# Autodesk Inventor assembly: 라즈베리파이 조립품
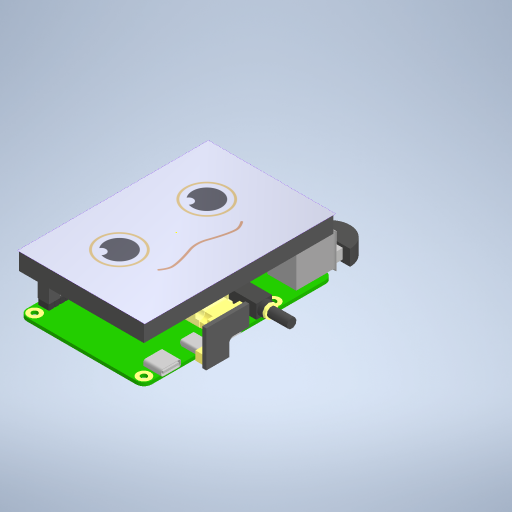
[picture p0: Inventor's stored thumbnail of the model, 512x512]
Saved by Autodesk Inventor 2023 (Build 270158000, 158)
## iProperties
Created: 2022-08-09
Part Number: 라즈베리파이 조립품
Document SubType Name: Assembly
Designer: fly01
Author: fly01
## Documents named in this file (6)
- C:\Users\user\Desktop\PAI\PAI설계\조림품\라즈베리파이 조립품.iam
- C:\Users\user\Desktop\PAI\PAI설계\범용 부품\raspberry.ipt
- C:\Users\user\Desktop\PAI\PAI설계\범용 부품\lcd 디스플레이.ipt
- C:\Users\user\Desktop\PAI\PAI설계\범용 부품\HDMI_Port.ipt
- C:\Users\user\Desktop\PAI\PAI설계\범용 부품\Audio_jac.ipt
- C:\Users\user\Desktop\PAI\PAI설계\범용 부품\Mic.ipt
## Components (5 placed, 5 different names)
1. lcd 디스플레이:1 — 회전:1, 회전:2
2. raspberry:1 — 회전:1, 강체:1, 회전:3
3. HDMI_Port:1 — 회전:2
4. Audio_jac:1 — 강체:1
5. Mic:1 — 회전:3
## Relationships (4: RevoluteJoint 3, WeldJoint 1)
- 회전:1 [RevoluteJoint]: lcd 디스플레이:1 ↔ raspberry:1
- 회전:2 [RevoluteJoint] (-7.4 mm): lcd 디스플레이:1 ↔ HDMI_Port:1
- 강체:1 [WeldJoint]: raspberry:1 ↔ Audio_jac:1
- 회전:3 [RevoluteJoint] (3.9 mm): raspberry:1 ↔ Mic:1
